# Autodesk Inventor assembly: cooler_plate
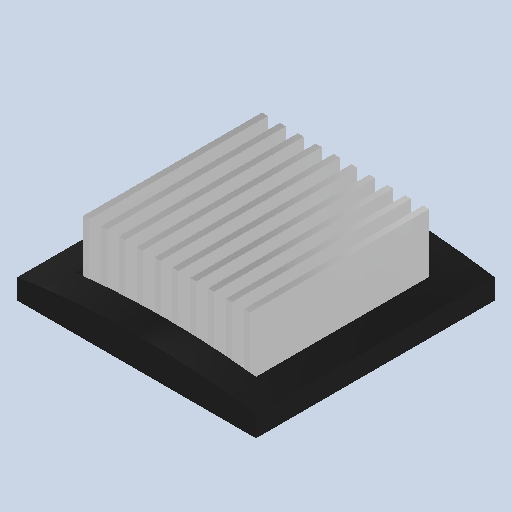
[picture p0: Inventor's stored thumbnail of the model, 512x512]
Saved by Autodesk Inventor 2023 (Build 270158000, 158)
## iProperties
Created: 2023-10-18
Part Number: cooler_plate
Document SubType Name: Assembly
Designer: 310611102
Author: 310611102
## Documents named in this file (3)
- C:\Users\310611102\Documents\Inventor\SSR\avionics_2023ver\assembly\cooler_plate_assemb.iam
- C:\Users\310611102\Documents\Inventor\SSR\avionics_2023ver\assembly\cooler_plate.ipt
- C:\Users\310611102\Documents\Inventor\SSR\avionics_2023ver\assembly\cooler_plate_socket.ipt
## Components (2 placed, 2 different names)
1. cooler_plate:1 — Mate:1, Mate:2
2. cooler_plate_socket:1 — Mate:1, Mate:2
## Relationships (2: Mate 2)
- Mate:1: cooler_plate:1 ↔ cooler_plate_socket:1
- Mate:2: cooler_plate:1 ↔ cooler_plate_socket:1
